# Autodesk Inventor assembly: pololuAssembly
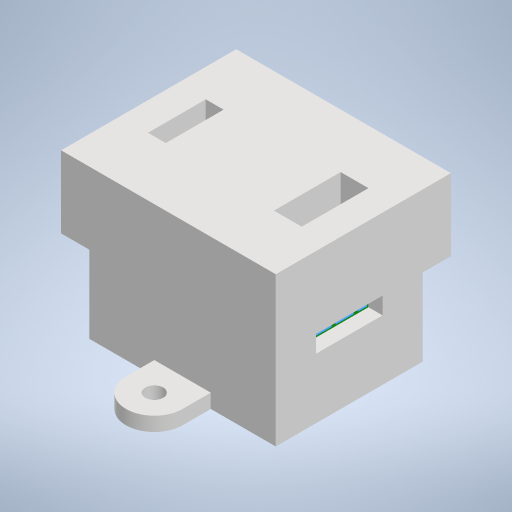
[picture p0: Inventor's stored thumbnail of the model, 512x512]
Saved by Autodesk Inventor 2024 (Build 280153000, 153)
## iProperties
Created: 2023-08-07
Part Number: pololuAssembly
Document SubType Name: Assembly
Designer: 18179
Author: 18179
## Documents named in this file (4)
- C:\Users\18179\Desktop\TuppyMkIV\pololuAssembly.iam
- C:\Users\18179\Desktop\TuppyMkIV\pololu-rc-switch-with-relay.ipt
- C:\Users\18179\Desktop\TuppyMkIV\pololuCaseBottom.ipt
- C:\Users\18179\Desktop\TuppyMkIV\pololuCaseTop.ipt
## Components (3 placed, 3 different names)
1. pololu-rc-switch-with-relay:1 — Mate:1, Mate:2, Mate:3
2. pololuCaseBottom:1 — Mate:1, Mate:2, Mate:3, Mate:4, Mate:5, Mate:6
3. pololuCaseTop:1 — Mate:4, Mate:5, Mate:6
## Relationships (6: Mate 6)
- Mate:1: pololu-rc-switch-with-relay:1 ↔ pololuCaseBottom:1
- Mate:2: pololu-rc-switch-with-relay:1 ↔ pololuCaseBottom:1
- Mate:3: pololu-rc-switch-with-relay:1 ↔ pololuCaseBottom:1
- Mate:4: pololuCaseBottom:1 ↔ pololuCaseTop:1
- Mate:5: pololuCaseBottom:1 ↔ pololuCaseTop:1
- Mate:6: pololuCaseBottom:1 ↔ pololuCaseTop:1
